# Autodesk Inventor assembly: ASY WRS АБК
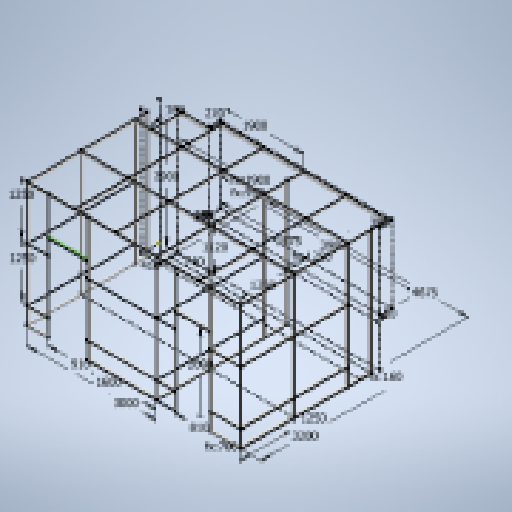
[picture p0: Inventor's stored thumbnail of the model, 512x512]
Saved by Autodesk Inventor 2024.2 (Build 282272000, 272)
## iProperties
_SolveAssemblyDoc: Frame Generator Solve Assembly
_Version: 25.0.0
Created: 2024-04-09
Part Number: ASY WRS АБК
Document SubType Name: Assembly
Designer: admin
Author: admin
## Documents named in this file (4)
- C:\Users\admin\My Drive (bigstupidbeast@gmail.com)\Inventor\Workshop\ASY WRS АБК.iam
- C:\Users\admin\My Drive (bigstupidbeast@gmail.com)\Inventor\Workshop\бытовка.ipt
- C:\Users\admin\My Drive (bigstupidbeast@gmail.com)\Inventor\Workshop\ASY WRS АБК\Frame\Frame 1712678974957.iam
- C:\Users\admin\My Drive (bigstupidbeast@gmail.com)\Inventor\Workshop\OSB плита\1250х2500Х18.ipt
## Components (8 placed, 3 different names)
1. бытовка:1 — Flush:1, Flush:2, Flush:3
2. Frame 1712678974957:1 [sub-assembly]
3. 1250х2500Х18:1 — Rigid:1, Rigid:3
4. 1250х2500Х18:2 — Rigid:1, Rigid:2, Rigid:4
5. 1250х2500Х18:3 — Rigid:2, Rigid:5
6. 1250х2500Х18:4 — Rigid:4
7. 1250х2500Х18:5 — Rigid:5
8. 1250х2500Х18:6 — Rigid:3
## Relationships (8: WeldJoint 5, Flush 3)
- Flush:1: бытовка:1
- Flush:2: бытовка:1
- Flush:3: бытовка:1
- Rigid:1 [WeldJoint]: 1250х2500Х18:1 ↔ 1250х2500Х18:2
- Rigid:2 [WeldJoint]: 1250х2500Х18:2 ↔ 1250х2500Х18:3
- Rigid:3 [WeldJoint]: 1250х2500Х18:1 ↔ 1250х2500Х18:6
- Rigid:4 [WeldJoint]: 1250х2500Х18:2 ↔ 1250х2500Х18:4
- Rigid:5 [WeldJoint]: 1250х2500Х18:3 ↔ 1250х2500Х18:5
